# Autodesk Inventor assembly: 110033226_iam_06_城堡四角塔
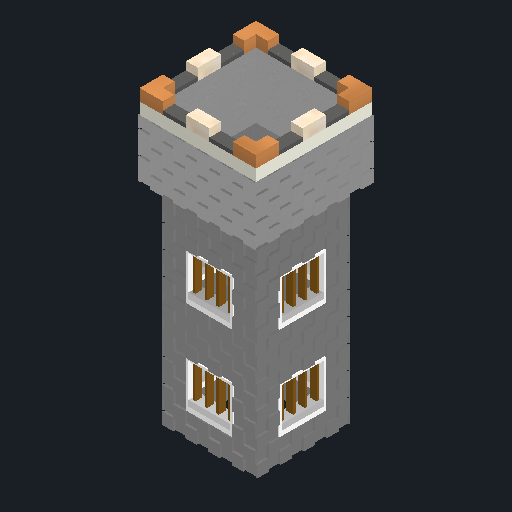
[picture p0: Inventor's stored thumbnail of the model, 512x512]
Saved by Autodesk Inventor 2022 (Build 260153000, 153)
## iProperties
Created: 2022-06-24
Part Number: 110033226_iam_06_城堡四角塔
Document SubType Name: Assembly
Designer: User
Author: User
## Documents named in this file (7)
- D:\D-disk\pomelo\大一\下學期\機械設計製圖\1100332260_LEGOproj_沒有公主城堡\110033226_iam_06_城堡四角塔.iam
- D:\D-disk\pomelo\大一\下學期\機械設計製圖\1100332260_LEGOproj_沒有公主城堡\110033226_ipt_28_城堡四圓塔.ipt
- D:\D-disk\pomelo\大一\下學期\機械設計製圖\1100332260_LEGOproj_沒有公主城堡\110033226_ipt_29_城堡四圓塔的窗戶.ipt
- D:\D-disk\pomelo\大一\下學期\機械設計製圖\1100332260_LEGOproj_沒有公主城堡\110033226_ipt_30_城堡四圓塔的頂部.ipt
- D:\D-disk\pomelo\大一\下學期\機械設計製圖\1100332260_LEGOproj_沒有公主城堡\110033226_ipt_12_平滑面(2x1).ipt
- D:\D-disk\pomelo\大一\下學期\機械設計製圖\1100332260_LEGOproj_沒有公主城堡\110033226_ipt_31_城堡四圓塔的頂部角落.ipt
- D:\D-disk\pomelo\大一\下學期\機械設計製圖\1100332260_LEGOproj_沒有公主城堡\110033226_ipt_32_平滑木塊(2x1).ipt
## Components (26 placed, 6 different names)
1. 110033226_ipt_28_城堡四圓塔:1 — 貼合:1, 貼合:2, 貼合:3, 貼合:4, 貼合:5, 貼合:6, 貼合:7, 貼合:8, 貼合:9
2. 110033226_ipt_30_城堡四圓塔的頂部:1 — 貼合:7, 貼合:8, 貼合:9, 貼合:10, 貼合:11, 貼合:12, 貼合:13, 貼合:14, 貼合:15, 貼合:16, 貼合:17
3. 110033226_ipt_31_城堡四圓塔的頂部角落:1 — 貼合:13, 貼合:14, 貼合:15
4. 110033226_ipt_31_城堡四圓塔的頂部角落:2
5. 110033226_ipt_31_城堡四圓塔的頂部角落:3
6. 110033226_ipt_31_城堡四圓塔的頂部角落:4
7. 110033226_ipt_32_平滑木塊(2x1):1 — 貼合:16, 貼合:17
8. 110033226_ipt_32_平滑木塊(2x1):2
9. 110033226_ipt_32_平滑木塊(2x1):3
10. 110033226_ipt_32_平滑木塊(2x1):4
11. 110033226_ipt_29_城堡四圓塔的窗戶:1 — 貼合:4, 貼合:5, 貼合:6
12. 110033226_ipt_29_城堡四圓塔的窗戶:2
13. 110033226_ipt_29_城堡四圓塔的窗戶:3
14. 110033226_ipt_29_城堡四圓塔的窗戶:4
15. 110033226_ipt_29_城堡四圓塔的窗戶:5
16. 110033226_ipt_29_城堡四圓塔的窗戶:6
17. 110033226_ipt_29_城堡四圓塔的窗戶:7
18. 110033226_ipt_29_城堡四圓塔的窗戶:8
19. 110033226_ipt_12_平滑面(2x1):1 — 貼合:10, 貼合:11, 貼合:12
20. 110033226_ipt_12_平滑面(2x1):5
21. 110033226_ipt_12_平滑面(2x1):6
22. 110033226_ipt_12_平滑面(2x1):7
23. 110033226_ipt_12_平滑面(2x1):8
24. 110033226_ipt_12_平滑面(2x1):9
25. 110033226_ipt_12_平滑面(2x1):10
26. 110033226_ipt_12_平滑面(2x1):11
## Component patterns: (2 elements), (4 elements), (4 elements, first: 110033226_ipt_31_城堡四圓塔的頂部角落:1), (4 elements, first: 110033226_ipt_32_平滑木塊(2x1):1), (4 elements, first: 110033226_ipt_29_城堡四圓塔的窗戶:1), 元件陣列 1:2 (4 elements), (2 elements, first: 110033226_ipt_12_平滑面(2x1):1), 元件陣列 3:2 (2 elements), 元件陣列 3:3 (2 elements), 元件陣列 3:4 (2 elements)
## Relationships (17: Mate 17)
- 貼合:1 [Mate]: 110033226_ipt_28_城堡四圓塔:1
- 貼合:2 [Mate]: 110033226_ipt_28_城堡四圓塔:1
- 貼合:3 [Mate]: 110033226_ipt_28_城堡四圓塔:1
- 貼合:4 [Mate]: 110033226_ipt_28_城堡四圓塔:1 ↔ 110033226_ipt_29_城堡四圓塔的窗戶:1
- 貼合:5 [Mate]: 110033226_ipt_28_城堡四圓塔:1 ↔ 110033226_ipt_29_城堡四圓塔的窗戶:1
- 貼合:6 [Mate]: 110033226_ipt_28_城堡四圓塔:1 ↔ 110033226_ipt_29_城堡四圓塔的窗戶:1
- 貼合:7 [Mate]: 110033226_ipt_28_城堡四圓塔:1 ↔ 110033226_ipt_30_城堡四圓塔的頂部:1
- 貼合:8 [Mate]: 110033226_ipt_28_城堡四圓塔:1 ↔ 110033226_ipt_30_城堡四圓塔的頂部:1
- 貼合:9 [Mate]: 110033226_ipt_28_城堡四圓塔:1 ↔ 110033226_ipt_30_城堡四圓塔的頂部:1
- 貼合:10 [Mate]: 110033226_ipt_30_城堡四圓塔的頂部:1 ↔ 110033226_ipt_12_平滑面(2x1):1
- 貼合:11 [Mate]: 110033226_ipt_30_城堡四圓塔的頂部:1 ↔ 110033226_ipt_12_平滑面(2x1):1
- 貼合:12 [Mate]: 110033226_ipt_30_城堡四圓塔的頂部:1 ↔ 110033226_ipt_12_平滑面(2x1):1
- 貼合:13 [Mate]: 110033226_ipt_30_城堡四圓塔的頂部:1 ↔ 110033226_ipt_31_城堡四圓塔的頂部角落:1
- 貼合:14 [Mate]: 110033226_ipt_30_城堡四圓塔的頂部:1 ↔ 110033226_ipt_31_城堡四圓塔的頂部角落:1
- 貼合:15 [Mate]: 110033226_ipt_30_城堡四圓塔的頂部:1 ↔ 110033226_ipt_31_城堡四圓塔的頂部角落:1
- 貼合:16 [Mate]: 110033226_ipt_30_城堡四圓塔的頂部:1 ↔ 110033226_ipt_32_平滑木塊(2x1):1
- 貼合:17 [Mate]: 110033226_ipt_30_城堡四圓塔的頂部:1 ↔ 110033226_ipt_32_平滑木塊(2x1):1
